# Autodesk Inventor assembly: Deltabot - Small Model
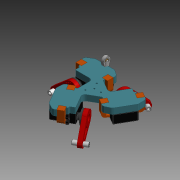
[picture p0: Inventor's stored thumbnail of the model, 180x180]
Saved by Autodesk Inventor 2014 SP1 (Build 180222100, 222)
## iProperties
Created: 2013-12-25
Part Number: Deltabot - Small Model
Document SubType Name: Assembly
Designer: tom
Title: D:\My Documents\Work\GitHub\Delta_Robots\Delatabot - Small Model\Deltabot - Small Model.stp
Creation Date: 2013-12-24
Sending System: ACIS
Author: tom
## Documents named in this file (6)
- C:\Users\tom\Documents\GitHub\Delta_Robots\Delatabot - Small Model\Imported Components\Deltabot - Small Model\Deltabot - Small Model.iam
- C:\Users\tom\Documents\GitHub\Delta_Robots\Delatabot - Small Model\Imported Components\Deltabot - Small Model\Component8 Copy2.ipt
- C:\Users\tom\Documents\GitHub\Delta_Robots\Delatabot - Small Model\Imported Components\Deltabot - Small Model\Servo Mechanism.iam
- C:\Users\tom\Documents\GitHub\Delta_Robots\Delatabot - Small Model\Imported Components\Deltabot - Small Model\Upper Arm.iam
- C:\Users\tom\Documents\GitHub\Delta_Robots\Delatabot - Small Model\Imported Components\Deltabot - Small Model\Bearing.ipt
- C:\Users\tom\Documents\GitHub\Delta_Robots\Delatabot - Small Model\Imported Components\Deltabot - Small Model\Body.ipt
## Components (9 placed, 5 different names)
1. Servo Plate — Mate:1, Mate:2, Mate:3, Mate:4, Mate:5, Mate:6, Mate:7, Mate:8, Mate:9
2. Servo Mechanism:1 [sub-assembly] — Mate:1, Mate:2, Mate:3, Rotational:1
3. Upper Arm:1 [sub-assembly] — Rotational:1
4. Servo Mechanism:2 [sub-assembly] — Mate:4, Mate:5, Mate:6, Rotational:2
5. Upper Arm:2 [sub-assembly] — Rotational:2
6. Servo Mechanism:3 [sub-assembly] — Mate:7, Mate:8, Mate:9, Rotational:3
7. Upper Arm:3 [sub-assembly] — Rotational:3
8. Bearing:1 — Flush:1
9. Body:1 — Flush:2
## Relationships (14: Mate 9, RevoluteJoint 3, Flush 2)
- Mate:1: Servo Plate ↔ Servo Mechanism:1
- Mate:2: Servo Plate ↔ Servo Mechanism:1
- Mate:3: Servo Plate ↔ Servo Mechanism:1
- Mate:4: Servo Plate ↔ Servo Mechanism:2
- Mate:5: Servo Plate ↔ Servo Mechanism:2
- Mate:6: Servo Plate ↔ Servo Mechanism:2
- Mate:7: Servo Plate ↔ Servo Mechanism:3
- Mate:8: Servo Plate ↔ Servo Mechanism:3
- Mate:9: Servo Plate ↔ Servo Mechanism:3
- Rotational:1 [RevoluteJoint]: Servo Mechanism:1 ↔ Upper Arm:1
- Rotational:2 [RevoluteJoint]: Servo Mechanism:2 ↔ Upper Arm:2
- Rotational:3 [RevoluteJoint]: Servo Mechanism:3 ↔ Upper Arm:3
- Flush:1: Bearing:1
- Flush:2: Body:1
